# Autodesk Inventor assembly: NEW Vertical Wing
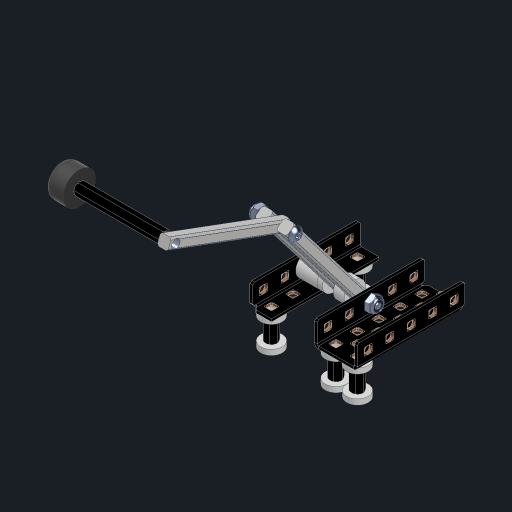
[picture p0: Inventor's stored thumbnail of the model, 512x512]
Saved by Autodesk Inventor 2023.2 (Build 272271030, 271C)
## iProperties
Created: 2024-02-11
Part Number: NEW Vertical Wing
Document SubType Name: Assembly
Designer: Michael
Author: Michael
## Documents named in this file (18)
- C:\Users\black\OneDrive\Pictures\Documents\GitHub\New folder\2024-599Z\Cad\NEW Wings\NEW Vertical Wing.iam
- C:\Users\black\OneDrive\Pictures\Documents\GitHub\New folder\2024-599Z\Cad\Library\VEX-CAD-Inventor-1.4.0\Structure\C Channel\Aluminum 1x2x1\Alu C 1x2x1x5.ipt
- C:\Users\black\OneDrive\Pictures\Documents\GitHub\New folder\2024-599Z\Cad\Library\VEX-CAD-Inventor-1.4.0\Structure\C Channel\Aluminum 1x3x1 Half\Alu C Half 1x3x1x5.ipt
- C:\Users\black\OneDrive\Pictures\Documents\GitHub\New folder\2024-599Z\Cad\Library\VEX-CAD-Inventor-1.4.0\Motion\Spacers\Spacer Nylon .500 OD\NSpacer White .500 OD x .500.ipt
- C:\Users\black\OneDrive\Pictures\Documents\GitHub\New folder\2024-599Z\Cad\Library\VEX-CAD-Inventor-1.4.0\Motion\Spacers\Spacer Nylon .500 OD.ipt
- C:\Users\black\OneDrive\Pictures\Documents\GitHub\New folder\2024-599Z\Cad\Library\VEX-CAD-Inventor-1.4.0\Motion\Spacers\Spacer Nylon .500 OD\NSpacer White .500 OD x .125.ipt
- C:\Users\black\OneDrive\Pictures\Documents\GitHub\New folder\2024-599Z\Cad\NEW Wings\Vertical Wing Shaft.iam
- C:\Users\black\OneDrive\Pictures\Documents\GitHub\New folder\2024-599Z\Cad\Library\VEX-CAD-Inventor-1.4.0\Motion\Spacers\Spacer Nylon .500 OD\NSpacer White .500 OD x .250.ipt
- C:\Users\black\OneDrive\Pictures\Documents\GitHub\New folder\2024-599Z\Cad\Library\VEX-CAD-Inventor-1.4.0\Motion\Spacers\Washer Teflon\TWasher .375 OD x .06250.ipt
- C:\Users\black\OneDrive\Pictures\Documents\GitHub\New folder\2024-599Z\Cad\Library\VEX-CAD-Inventor-1.4.0\Motion\Spacers\Washer Teflon.ipt
- C:\Users\black\OneDrive\Pictures\Documents\GitHub\New folder\2024-599Z\Cad\Library\VEX-CAD-Inventor-1.4.0\Structure\Hardware\Screw Steel - Star\SScrew Star Smooth 1.750.ipt
- C:\Users\black\OneDrive\Pictures\Documents\GitHub\New folder\2024-599Z\Cad\Library\VEX-CAD-Inventor-1.4.0\Structure\Hardware\Screw Steel - Star.ipt
- C:\Users\black\OneDrive\Pictures\Documents\GitHub\New folder\2024-599Z\Cad\Library\VEX-CAD-Inventor-1.4.0\Structure\Hardware\Screw Steel - Star\SScrew Star Smooth 1.000.ipt
- C:\Users\black\OneDrive\Pictures\Documents\GitHub\New folder\2024-599Z\Cad\Library\VEX-CAD-Inventor-1.4.0\Structure\Hardware\Nut Thin Nylock.ipt
- C:\Users\black\OneDrive\Pictures\Documents\GitHub\New folder\2024-599Z\Cad\Library\VEX-CAD-Inventor-1.4.0\Structure\Standoff\Standoff 2.00.ipt
- C:\Users\black\OneDrive\Pictures\Documents\GitHub\New folder\2024-599Z\Cad\Library\VEX-CAD-Inventor-1.4.0\Structure\Standoff.ipt
- C:\Users\black\OneDrive\Pictures\Documents\GitHub\New folder\2024-599Z\Cad\Library\VEX-CAD-Inventor-1.4.0\Structure\Standoff\Standoff .50.ipt
- C:\Users\black\OneDrive\Pictures\Documents\GitHub\New folder\2024-599Z\Cad\Library\VEX-CAD-Inventor-1.4.0\Structure\Hardware\Rubber Bumper Threaded.ipt
## Components (27 placed, 13 different names)
1. Alu C 1x2x1x5:1 — Insert:11, Insert:17, Insert:33, Insert:34
2. Alu C Half 1x3x1x5:2 — Insert:5, Insert:14, Insert:31, Insert:32
3. NSpacer White .500 OD x .500:1 — Insert:5, Insert:6
4. NSpacer White .500 OD x .125:2 — Insert:6, Insert:7
5. Vertical Wing Shaft:1 [sub-assembly] — Insert:7, Insert:8, Insert:13, Insert:16
6. Vertical Wing Shaft:2 [sub-assembly] — Insert:9, Insert:10, Insert:12, Insert:15
7. NSpacer White .500 OD x .250:3 — Insert:8, Insert:9
8. TWasher .375 OD x .06250:1 — Insert:10, Insert:11
9. Vertical Wing Shaft:3 [sub-assembly] — Insert:12, Insert:13, Insert:21
10. SScrew Star Smooth 1.750:1 — Insert:14
11. SScrew Star Smooth 1.000:2 — Insert:15
12. Nut Thin Nylock:1 — Insert:16
13. Nut Thin Nylock:2 — Insert:17
14. Standoff 2.00:3 — Insert:21, Insert:22
15. Rubber Bumper Threaded:1 — Insert:22
16. Standoff .50:6 — Insert:23, Insert:24
17. NSpacer White .500 OD x .125:5 — Insert:23, Insert:31
18. NSpacer White .500 OD x .125:6 — Insert:24
19. Standoff .50:7
20. NSpacer White .500 OD x .125:7 — Insert:32
21. NSpacer White .500 OD x .125:8
22. Standoff .50:8
23. NSpacer White .500 OD x .125:9 — Insert:33
24. NSpacer White .500 OD x .125:10
25. Standoff .50:9
26. NSpacer White .500 OD x .125:11 — Insert:34
27. NSpacer White .500 OD x .125:12
## Relationships (27: Insert 27)
- Insert:5: Alu C Half 1x3x1x5:2 ↔ NSpacer White .500 OD x .500:1
- Insert:6: NSpacer White .500 OD x .500:1 ↔ NSpacer White .500 OD x .125:2
- Insert:7: NSpacer White .500 OD x .125:2 ↔ Vertical Wing Shaft:1
- Insert:8: Vertical Wing Shaft:1 ↔ NSpacer White .500 OD x .250:3
- Insert:9: Vertical Wing Shaft:2 ↔ NSpacer White .500 OD x .250:3
- Insert:10: Vertical Wing Shaft:2 ↔ TWasher .375 OD x .06250:1
- Insert:11: Alu C 1x2x1x5:1 ↔ TWasher .375 OD x .06250:1
- Insert:12: Vertical Wing Shaft:2 ↔ Vertical Wing Shaft:3
- Insert:13: Vertical Wing Shaft:1 ↔ Vertical Wing Shaft:3
- Insert:14: Alu C Half 1x3x1x5:2 ↔ SScrew Star Smooth 1.750:1
- Insert:15: Vertical Wing Shaft:2 ↔ SScrew Star Smooth 1.000:2
- Insert:16: Vertical Wing Shaft:1 ↔ Nut Thin Nylock:1
- Insert:17: Alu C 1x2x1x5:1 ↔ Nut Thin Nylock:2
- Insert:21: Vertical Wing Shaft:3 ↔ Standoff 2.00:3
- Insert:22: Standoff 2.00:3 ↔ Rubber Bumper Threaded:1
- Insert:23: Standoff .50:6 ↔ NSpacer White .500 OD x .125:5
- Insert:24: Standoff .50:6 ↔ NSpacer White .500 OD x .125:6
- [Insert]: Standoff .50:7 ↔ NSpacer White .500 OD x .125:7
- [Insert]: Standoff .50:7 ↔ NSpacer White .500 OD x .125:8
- [Insert]: Standoff .50:8 ↔ NSpacer White .500 OD x .125:9
- [Insert]: Standoff .50:8 ↔ NSpacer White .500 OD x .125:10
- [Insert]: Standoff .50:9 ↔ NSpacer White .500 OD x .125:11
- [Insert]: Standoff .50:9 ↔ NSpacer White .500 OD x .125:12
- Insert:31: Alu C Half 1x3x1x5:2 ↔ NSpacer White .500 OD x .125:5
- Insert:32: Alu C Half 1x3x1x5:2 ↔ NSpacer White .500 OD x .125:7
- Insert:33: Alu C 1x2x1x5:1 ↔ NSpacer White .500 OD x .125:9
- Insert:34: Alu C 1x2x1x5:1 ↔ NSpacer White .500 OD x .125:11
## Named parameters: d26_d24 = 0 mm, d27_d25 = 0 mm, d28_d24 = 0 mm, d29_d25 = 0 mm, d30_d24 = 0 mm, d31_d25 = 0 mm
